# Autodesk Inventor assembly: Shooter v2 9-12-2020
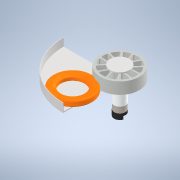
[picture p0: Inventor's stored thumbnail of the model, 180x180]
Saved by Autodesk Inventor 2021 (Build 250183000, 183)
## iProperties
Created: 2020-09-12
Part Number: Shooter v2 9-12-2020
Document SubType Name: Assembly
Designer: deli
Author: deli
## Documents named in this file (6)
- C:\Users\deli\OneDrive - Eastside Preparatory School\FTC\Ultamite Goal\Shooter v2 9-12-2020.iam
- C:\Users\deli\OneDrive - Eastside Preparatory School\FTC\Ultamite Goal\ramp.ipt
- C:\Users\deli\OneDrive - Eastside Preparatory School\FTC\Ultamite Goal\5_ Straight Flex Wheel (30A) (217-6453).ipt
- C:\Users\deli\OneDrive - Eastside Preparatory School\FTC\Ultamite Goal\5inCompliantWheelHub.ipt
- C:\Users\deli\OneDrive - Eastside Preparatory School\FTC\Ultamite Goal\am-3461a NeveRest 4 with Motor REV3.ipt
- C:\Users\deli\OneDrive - Eastside Preparatory School\FTC\Ultamite Goal\am-4300 Ring.ipt
## Components (5 placed, 5 different names)
1. ramp:1 — Mate:5, Angle:1, Mate:6, Mate:8, Mate:9, Mate:10
2. 5_ Straight Flex Wheel (30A) (217-6453):1 — Mate:2, Mate:3, Mate:4
3. 5inCompliantWheelHub:1 — Mate:2, Mate:3, Mate:4, Mate:7, Mate:8
4. am-3461a NeveRest 4 with Motor REV3:1 — Mate:5, Angle:1, Mate:6, Mate:7
5. am-4300 Ring:1 — Mate:9, Mate:10
## Relationships (10: Mate 9, Angle 1)
- Mate:2: 5_ Straight Flex Wheel (30A) (217-6453):1 ↔ 5inCompliantWheelHub:1
- Mate:3: 5_ Straight Flex Wheel (30A) (217-6453):1 ↔ 5inCompliantWheelHub:1
- Mate:4: 5_ Straight Flex Wheel (30A) (217-6453):1 ↔ 5inCompliantWheelHub:1
- Mate:5: ramp:1 ↔ am-3461a NeveRest 4 with Motor REV3:1
- Angle:1 (0 deg): ramp:1 ↔ am-3461a NeveRest 4 with Motor REV3:1
- Mate:6: ramp:1 ↔ am-3461a NeveRest 4 with Motor REV3:1
- Mate:7: 5inCompliantWheelHub:1 ↔ am-3461a NeveRest 4 with Motor REV3:1
- Mate:8: ramp:1 ↔ 5inCompliantWheelHub:1
- Mate:9 (120.65 mm): ramp:1 ↔ am-4300 Ring:1
- Mate:10: ramp:1 ↔ am-4300 Ring:1
